# Autodesk Inventor assembly: StereoCabinet
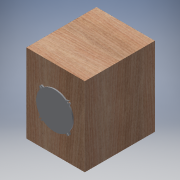
[picture p0: Inventor's stored thumbnail of the model, 180x180]
Saved by Autodesk Inventor 2017 (Build 210142000, 142)
## iProperties
Created: 2018-07-25
Part Number: StereoCabinet
Document SubType Name: Assembly
Designer: Jake
Author: Jake
## Documents named in this file (3)
- C:\Users\Jake\git\CAD-Projects\parts\Stereo\StereoCabinet.iam
- C:\Users\Jake\git\CAD-Projects\parts\Stereo\speakerBox.ipt
- C:\Users\Jake\git\CAD-Projects\parts\Stereo\speaker.ipt
## Components (2 placed, 2 different names)
1. speakerBox:1 — Rotational:1
2. speaker:1 — Rotational:1
## Relationships (1: RevoluteJoint 1)
- Rotational:1 [RevoluteJoint]: speakerBox:1 ↔ speaker:1
